# Autodesk Inventor assembly: lift_v2
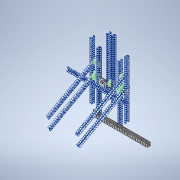
[picture p0: Inventor's stored thumbnail of the model, 180x180]
Saved by Autodesk Inventor 2021 (Build 250183000, 183)
## iProperties
Created: 2020-05-18
Part Number: lift_v2
Document SubType Name: Assembly
Designer: ajcar
Author: ajcar
## Documents named in this file (17)
- C:\Users\ajcar\Documents\vex_cad\lift\lift_v2.iam
- C:\Users\ajcar\Documents\vex_cad\lib\Team 7479 Solidworks Library\Structure\C-Channel\C-Channel 1x2x1x35.ipt
- C:\Users\ajcar\Documents\vex_cad\lib\Structure\2x2x35_Steel_Angle_275-1143.ipt
- C:\Users\ajcar\Documents\vex_cad\lib\Team 7479 Solidworks Library\Hardware\Bearings\Bearing Flat.ipt
- C:\Users\ajcar\Documents\vex_cad\lib\Team 7479 Solidworks Library\Hardware\Washers & Spacers\Nylon Spacer .5 .125in.ipt
- C:\Users\ajcar\Documents\vex_cad\lib\Team 7479 Solidworks Library\Hardware\Washers & Spacers\Teflon Washer.ipt
- C:\Users\ajcar\Documents\vex_cad\lib\Team 7479 Solidworks Library\Gears, Sprocket & Chain\High Strength Gears\Gear HS 36 Tooth.ipt
- C:\Users\ajcar\Documents\vex_cad\lib\Team 7479 Solidworks Library\Gears, Sprocket & Chain\High Strength Gears\Gear HS Insert Plastic.ipt
- C:\Users\ajcar\Documents\vex_cad\lib\Team 7479 Solidworks Library\Hardware\Screws & Nuts\Nuts\Nut 832 Keps.ipt
- C:\Users\ajcar\Documents\vex_cad\lib\Team 7479 Solidworks Library\Hardware\Screws & Nuts\Nuts\Nut 832 Nylock.ipt
- C:\Users\ajcar\Documents\vex_cad\lib\Team 7479 Solidworks Library\Gears, Sprocket & Chain\High Strength Gears\Gear HS 60 Tooth.ipt
- C:\Users\ajcar\Documents\vex_cad\lib\Team 7479 Solidworks Library\Hardware\Washers & Spacers\Nylon Spacer .5 .375in.ipt
- C:\Users\ajcar\Documents\vex_cad\lib\Team 7479 Solidworks Library\Electronics\Motors & Servos\V5_Smart_Motor_276-4840.ipt
- C:\Users\ajcar\Documents\vex_cad\lib\Team 7479 Solidworks Library\Gears, Sprocket & Chain\High Strength Gears\Gear HS 12 Tooth.ipt
- C:\Users\ajcar\Documents\vex_cad\lib\Team 7479 Solidworks Library\Hardware\Shafts\Shaft_Collar.ipt
- C:\Users\ajcar\Documents\vex_cad\lib\Team 7479 Solidworks Library\Hardware\Washers & Spacers\Steel Washer.ipt
- C:\Users\ajcar\Documents\vex_cad\lib\Team 7479 Solidworks Library\Hardware\Shafts\Drive Shaft 9.5-inches long.ipt
## Components (72 placed, 16 different names)
1. C-Channel 1x2x1x35:1 — Insert:124, Insert:125, Insert:132, Insert:144, Insert:145
2. C-Channel 1x2x1x35:2 — Insert:115, Insert:116, Insert:117, Insert:148, Insert:149
3. 2x2x35_Steel_Angle_275-1143:1
4. C-Channel 1x2x1x35:5 — Insert:113, Insert:114, Insert:150, Insert:151
5. C-Channel 1x2x1x35:6 — Insert:135, Insert:136, Insert:146, Insert:147
6. Bearing Flat:10
7. Bearing Flat:11
8. Gear HS 36 Tooth:1
9. Gear HS Insert Plastic:1
10. Gear HS Insert Plastic:2
11. Nut 832 Keps:1
12. Nut 832 Keps:2
13. Nut 832 Nylock:1
14. Nut 832 Nylock:2
15. C-Channel 1x2x1x35:9 — Angle:3
16. Nylon Spacer .5 .125in:31
17. Nylon Spacer .5 .125in:32
18. Gear HS 36 Tooth:2
19. Gear HS Insert Plastic:3
20. Gear HS Insert Plastic:4
21. C-Channel 1x2x1x35:10 — Angle:2
22. Bearing Flat:12 — Insert:113, Insert:114, Insert:187
23. Bearing Flat:13 — Insert:115, Insert:116
24. Nylon Spacer .5 .125in:33 — Insert:117, Insert:121
25. Gear HS 60 Tooth:1 — Insert:118, Insert:119, Insert:120
26. C-Channel 1x2x1x35:12 — Insert:118, Insert:119, Angle:2, Insert:122
27. Teflon Washer:1 — Insert:120, Insert:121
28. Nylon Spacer .5 .375in:1 — Insert:123
29. Nylon Spacer .5 .375in:2 — Insert:122, Insert:123
30. Bearing Flat:14 — Insert:124, Insert:125
31. Nylon Spacer .5 .125in:34 — Insert:132
32. Gear HS 60 Tooth:2
33. C-Channel 1x2x1x35:13 — Angle:3
34. Teflon Washer:2
35. Nylon Spacer .5 .375in:3
36. Nylon Spacer .5 .375in:4
37. Bearing Flat:15 — Insert:135, Insert:136
38. C-Channel 1x2x1x35:14 — Insert:138, Insert:139, Insert:140, Insert:143, Insert:164, Insert:165, Insert:169, Insert:175
39. V5_Smart_Motor_276-4840:1 — Insert:138, Insert:139
40. C-Channel 1x2x1x35:15 — Insert:141, Insert:142, Insert:167, Insert:168, Insert:178, Insert:179
41. Nylon Spacer .5 .125in:35 — Insert:140, Insert:158
42. Nylon Spacer .5 .125in:36 — Insert:142, Insert:156
43. Nylon Spacer .5 .125in:37 — Insert:141, Insert:157
44. Nylon Spacer .5 .125in:38 — Insert:143, Insert:159
45. Nylon Spacer .5 .125in:39 — Insert:147, Insert:161
46. Nylon Spacer .5 .125in:40 — Insert:145, Insert:162
47. Nylon Spacer .5 .125in:41 — Insert:144, Insert:163
48. Nylon Spacer .5 .125in:42 — Insert:146, Insert:160
49. Nylon Spacer .5 .125in:43 — Insert:148, Insert:155
50. Nylon Spacer .5 .125in:44 — Insert:149, Insert:154
51. Nylon Spacer .5 .125in:45 — Insert:151, Insert:153
52. Nylon Spacer .5 .125in:46 — Insert:150, Insert:152
53. C-Channel 1x2x1x35:16 — Insert:152, Insert:153, Insert:154, Insert:155, Insert:156, Insert:157, Insert:158, Insert:159, Insert:160, Insert:161, Insert:162, Insert:163
54. Bearing Flat:16 — Insert:164, Insert:165
55. Bearing Flat:17 — Insert:167, Insert:168
56. Gear HS 12 Tooth:1 — Insert:170, Insert:171
57. Teflon Washer:3 — Insert:169, Insert:170
58. Teflon Washer:4 — Insert:171, Insert:172
59. Shaft_Collar:1 — Insert:172, Insert:173
60. Teflon Washer:5 — Insert:173, Insert:174
61. Steel Washer:1 — Insert:174
62. Teflon Washer:6 — Insert:175, Insert:176
63. Gear HS 36 Tooth:3 — Insert:177, Insert:180
64. Teflon Washer:7 — Insert:176, Insert:177
65. Bearing Flat:18 — Insert:178, Insert:179
66. Teflon Washer:8 — Insert:180, Insert:181
67. Teflon Washer:9 — Insert:181, Insert:182
68. Shaft_Collar:2 — Insert:182, Insert:184
69. Teflon Washer:10 — Insert:184, Insert:185
70. Teflon Washer:11 — Insert:185, Insert:186
71. Steel Washer:2 — Insert:186
72. Drive Shaft 9.5-inches long:1 — Insert:187
## Relationships (98: Insert 92, Angle 3, Mate 2, Flush 1)
- [Mate]: C-Channel 1x2x1x35:1 ↔ 2x2x35_Steel_Angle_275-1143:1
- [Mate]: C-Channel 1x2x1x35:2 ↔ 2x2x35_Steel_Angle_275-1143:1
- [Angle] (0 deg): C-Channel 1x2x1x35:2 ↔ 2x2x35_Steel_Angle_275-1143:1
- [Insert]: C-Channel 1x2x1x35:1 ↔ 2x2x35_Steel_Angle_275-1143:1
- [Insert]: C-Channel 1x2x1x35:2 ↔ 2x2x35_Steel_Angle_275-1143:1
- [Insert]: C-Channel 1x2x1x35:1 ↔ Bearing Flat:10
- [Insert]: C-Channel 1x2x1x35:1 ↔ Bearing Flat:10
- [Insert]: C-Channel 1x2x1x35:2 ↔ Bearing Flat:11
- [Insert]: C-Channel 1x2x1x35:2 ↔ Bearing Flat:11
- [Insert]: Gear HS 36 Tooth:1 ↔ Gear HS Insert Plastic:2
- [Insert]: Gear HS 36 Tooth:1 ↔ Gear HS Insert Plastic:1
- [Insert]: C-Channel 1x2x1x35:1 ↔ Nut 832 Keps:1
- [Insert]: C-Channel 1x2x1x35:2 ↔ Nut 832 Keps:2
- [Insert]: Gear HS 36 Tooth:1 ↔ C-Channel 1x2x1x35:9
- [Insert]: Gear HS 36 Tooth:1 ↔ C-Channel 1x2x1x35:9
- [Insert]: C-Channel 1x2x1x35:9 ↔ Nylon Spacer .5 .125in:31
- [Insert]: Nut 832 Nylock:1 ↔ Nylon Spacer .5 .125in:31
- [Insert]: Gear HS 36 Tooth:2 ↔ Gear HS Insert Plastic:4
- [Insert]: Gear HS 36 Tooth:2 ↔ Gear HS Insert Plastic:3
- [Insert]: Nut 832 Keps:2 ↔ Gear HS Insert Plastic:3
- [Insert]: Gear HS 36 Tooth:2 ↔ C-Channel 1x2x1x35:10
- [Insert]: Gear HS 36 Tooth:2 ↔ C-Channel 1x2x1x35:10
- [Insert]: Nylon Spacer .5 .125in:32 ↔ C-Channel 1x2x1x35:10
- [Insert]: Nut 832 Nylock:2 ↔ Nylon Spacer .5 .125in:32
- [Flush]: C-Channel 1x2x1x35:9 ↔ C-Channel 1x2x1x35:10
- [Insert]: Gear HS Insert Plastic:1 ↔ Nut 832 Keps:1
- Insert:113: C-Channel 1x2x1x35:5 ↔ Bearing Flat:12
- Insert:114: C-Channel 1x2x1x35:5 ↔ Bearing Flat:12
- Insert:115: C-Channel 1x2x1x35:2 ↔ Bearing Flat:13
- Insert:116: C-Channel 1x2x1x35:2 ↔ Bearing Flat:13
- Insert:117: C-Channel 1x2x1x35:2 ↔ Nylon Spacer .5 .125in:33
- Insert:118: Gear HS 60 Tooth:1 ↔ C-Channel 1x2x1x35:12
- Insert:119: Gear HS 60 Tooth:1 ↔ C-Channel 1x2x1x35:12
- Insert:120: Gear HS 60 Tooth:1 ↔ Teflon Washer:1
- Insert:121: Nylon Spacer .5 .125in:33 ↔ Teflon Washer:1
- Angle:2 (180 deg): C-Channel 1x2x1x35:10 ↔ C-Channel 1x2x1x35:12
- Insert:122: C-Channel 1x2x1x35:12 ↔ Nylon Spacer .5 .375in:2
- Insert:123: Nylon Spacer .5 .375in:1 ↔ Nylon Spacer .5 .375in:2
- Insert:124: C-Channel 1x2x1x35:1 ↔ Bearing Flat:14
- Insert:125: C-Channel 1x2x1x35:1 ↔ Bearing Flat:14
- [Insert]: Gear HS 60 Tooth:2 ↔ C-Channel 1x2x1x35:13
- [Insert]: Gear HS 60 Tooth:2 ↔ C-Channel 1x2x1x35:13
- [Insert]: Gear HS 60 Tooth:2 ↔ Teflon Washer:2
- [Insert]: Nylon Spacer .5 .125in:34 ↔ Teflon Washer:2
- [Insert]: C-Channel 1x2x1x35:13 ↔ Nylon Spacer .5 .375in:4
- [Insert]: Nylon Spacer .5 .375in:3 ↔ Nylon Spacer .5 .375in:4
- Insert:132: C-Channel 1x2x1x35:1 ↔ Nylon Spacer .5 .125in:34
- Angle:3 (180 deg): C-Channel 1x2x1x35:9 ↔ C-Channel 1x2x1x35:13
- Insert:135: C-Channel 1x2x1x35:6 ↔ Bearing Flat:15
- Insert:136: C-Channel 1x2x1x35:6 ↔ Bearing Flat:15
- Insert:138: C-Channel 1x2x1x35:14 ↔ V5_Smart_Motor_276-4840:1
- Insert:139: C-Channel 1x2x1x35:14 ↔ V5_Smart_Motor_276-4840:1
- Insert:140: C-Channel 1x2x1x35:14 ↔ Nylon Spacer .5 .125in:35
- Insert:141: C-Channel 1x2x1x35:15 ↔ Nylon Spacer .5 .125in:37
- Insert:142: C-Channel 1x2x1x35:15 ↔ Nylon Spacer .5 .125in:36
- Insert:143: C-Channel 1x2x1x35:14 ↔ Nylon Spacer .5 .125in:38
- Insert:144: C-Channel 1x2x1x35:1 ↔ Nylon Spacer .5 .125in:41
- Insert:145: C-Channel 1x2x1x35:1 ↔ Nylon Spacer .5 .125in:40
- Insert:146: C-Channel 1x2x1x35:6 ↔ Nylon Spacer .5 .125in:42
- Insert:147: C-Channel 1x2x1x35:6 ↔ Nylon Spacer .5 .125in:39
- Insert:148: C-Channel 1x2x1x35:2 ↔ Nylon Spacer .5 .125in:43
- Insert:149: C-Channel 1x2x1x35:2 ↔ Nylon Spacer .5 .125in:44
- Insert:150: C-Channel 1x2x1x35:5 ↔ Nylon Spacer .5 .125in:46
- Insert:151: C-Channel 1x2x1x35:5 ↔ Nylon Spacer .5 .125in:45
- Insert:152: Nylon Spacer .5 .125in:46 ↔ C-Channel 1x2x1x35:16
- Insert:153: Nylon Spacer .5 .125in:45 ↔ C-Channel 1x2x1x35:16
- Insert:154: Nylon Spacer .5 .125in:44 ↔ C-Channel 1x2x1x35:16
- Insert:155: Nylon Spacer .5 .125in:43 ↔ C-Channel 1x2x1x35:16
- Insert:156: Nylon Spacer .5 .125in:36 ↔ C-Channel 1x2x1x35:16
- Insert:157: Nylon Spacer .5 .125in:37 ↔ C-Channel 1x2x1x35:16
- Insert:158: Nylon Spacer .5 .125in:35 ↔ C-Channel 1x2x1x35:16
- Insert:159: Nylon Spacer .5 .125in:38 ↔ C-Channel 1x2x1x35:16
- Insert:160: Nylon Spacer .5 .125in:42 ↔ C-Channel 1x2x1x35:16
- Insert:161: Nylon Spacer .5 .125in:39 ↔ C-Channel 1x2x1x35:16
- Insert:162: Nylon Spacer .5 .125in:40 ↔ C-Channel 1x2x1x35:16
- Insert:163: Nylon Spacer .5 .125in:41 ↔ C-Channel 1x2x1x35:16
- Insert:164: C-Channel 1x2x1x35:14 ↔ Bearing Flat:16
- Insert:165: C-Channel 1x2x1x35:14 ↔ Bearing Flat:16
- Insert:167: C-Channel 1x2x1x35:15 ↔ Bearing Flat:17
- Insert:168: C-Channel 1x2x1x35:15 ↔ Bearing Flat:17
- Insert:169: C-Channel 1x2x1x35:14 ↔ Teflon Washer:3
- Insert:170: Gear HS 12 Tooth:1 ↔ Teflon Washer:3
- Insert:171: Gear HS 12 Tooth:1 ↔ Teflon Washer:4
- Insert:172: Teflon Washer:4 ↔ Shaft_Collar:1
- Insert:173: Shaft_Collar:1 ↔ Teflon Washer:5
- Insert:174: Teflon Washer:5 ↔ Steel Washer:1
- Insert:175: C-Channel 1x2x1x35:14 ↔ Teflon Washer:6
- Insert:176: Teflon Washer:6 ↔ Teflon Washer:7
- Insert:177: Gear HS 36 Tooth:3 ↔ Teflon Washer:7
- Insert:178: C-Channel 1x2x1x35:15 ↔ Bearing Flat:18
- Insert:179: C-Channel 1x2x1x35:15 ↔ Bearing Flat:18
- Insert:180: Gear HS 36 Tooth:3 ↔ Teflon Washer:8
- Insert:181: Teflon Washer:8 ↔ Teflon Washer:9
- Insert:182: Teflon Washer:9 ↔ Shaft_Collar:2
- Insert:184: Shaft_Collar:2 ↔ Teflon Washer:10
- Insert:185: Teflon Washer:10 ↔ Teflon Washer:11
- Insert:186: Teflon Washer:11 ↔ Steel Washer:2
- Insert:187: Bearing Flat:12 ↔ Drive Shaft 9.5-inches long:1
## Named parameters: d230_d218 = 0 mm, d231_d219 = 0 mm, d172_d166 = 0 mm, d173_d168 = 0 mm, d174_d169 = 0 mm, d175_d163 = 0 mm, d176_d164 = 0 mm, d177_d165 = 0 mm
